# Autodesk Inventor assembly: Hybrid
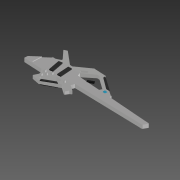
[picture p0: Inventor's stored thumbnail of the model, 180x180]
Saved by Autodesk Inventor 2020 (Build 240168000, 168)
## iProperties
Created: 2022-11-11
Part Number: Hybrid
Document SubType Name: Assembly
Designer: valer
Author: valer
## Documents named in this file (4)
- C:\Users\valer\Desktop\hybrid\src\Hybrid.iam
- C:\Users\valer\Desktop\hybrid\src\Hybrid.ipt
- C:\Users\valer\Desktop\hybrid\src\01BinaryLogo.ipt
- C:\Users\valer\Desktop\hybrid\src\OscilloscopeScreen.ipt
## Components (3 placed, 3 different names)
1. Hybrid:1 — Flush:1, Mate:1, Flush:2
2. 01BinaryLogo:1 — Flush:1, Mate:1
3. OscilloscopeScreen:1 — Flush:2
## Relationships (3: Flush 2, Mate 1)
- Flush:1 (-2 mm): Hybrid:1 ↔ 01BinaryLogo:1
- Mate:1: Hybrid:1 ↔ 01BinaryLogo:1
- Flush:2: Hybrid:1 ↔ OscilloscopeScreen:1
